# Autodesk Inventor assembly: slider
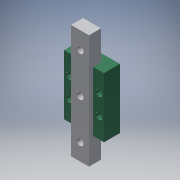
[picture p0: Inventor's stored thumbnail of the model, 180x180]
Saved by Autodesk Inventor 2018 (Build 220112000, 112)
## iProperties
Created: 2025-02-27
Part Number: slider
Document SubType Name: Assembly
Designer: neo
Author: neo
## Documents named in this file (3)
- C:\Users\neo\Documents\projects\kreion\design1\slider.iam
- C:\Users\neo\Documents\projects\kreion\design1\slider-rail.ipt
- C:\Users\neo\Documents\projects\kreion\design1\slider-slider.ipt
## Components (2 placed, 2 different names)
1. slider-rail:1 — Mate:1, Mate:2
2. slider-slider:1 — Mate:1, Mate:2
## Relationships (2: Mate 2)
- Mate:1: slider-rail:1 ↔ slider-slider:1
- Mate:2: slider-rail:1 ↔ slider-slider:1
